# Autodesk Inventor assembly: Z Drive Assembly
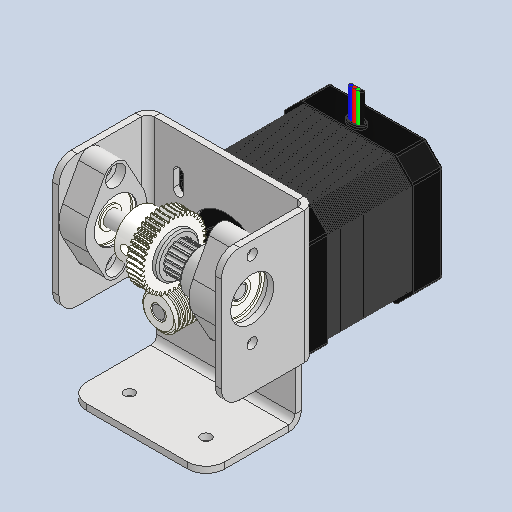
[picture p0: Inventor's stored thumbnail of the model, 512x512]
Saved by Autodesk Inventor 2022 (Build 260153000, 153)
## iProperties
Created: 2022-02-13
Part Number: Z Drive Assembly
Document SubType Name: Assembly
Designer: nicol
Author: nicol
## Documents named in this file (9)
- Z:\Projects\Bibble0\Z Drive Assembly.iam
- Z:\Projects\Bibble0\Sheet Metal\Z Drive Mount.ipt
- Z:\Projects\Bibble0\3D printed\Z Drive Bearing Holder.ipt
- Z:\Projects\Bibble0\Bearings\625 Bearing.ipt
- Z:\Projects\Bibble0\Hardware\5 x 50mm Shaft.ipt
- Z:\Projects\Bibble0\Hardware\GT2 Pulley 16T.ipt
- Z:\Projects\Bibble0\Hardware\METAL WORM GEAR_57545K624 v5.ipt
- Z:\Projects\Bibble0\Hardware\PLASTIC WORM GEAR_4037N115 v3.ipt
- Z:\Projects\Bibble0\Electronics\NEMA 17.ipt
## Components (10 placed, 8 different names)
1. Z Drive Mount:1 — Insert:4, Insert:5, Insert:6, Mate:5, Insert:8, Insert:9
2. Z Drive Bearing Holder:1 — Insert:4, Insert:5
3. Z Drive Bearing Holder:2 — Insert:6
4. 625 Bearing:1 — Mate:4
5. 625 Bearing:2
6. 5 x 50mm Shaft:1 — Mate:4
7. GT2 Pulley 16T:1
8. METAL WORM GEAR_57545K624 v5:1 — Insert:7
9. PLASTIC WORM GEAR_4037N115 v3:1
10. NEMA 17:1 — Mate:5, Insert:7, Insert:8, Insert:9
## Relationships (15: Insert 9, Mate 5, Flush 1)
- [Insert]: Z Drive Bearing Holder:2 ↔ 625 Bearing:1
- [Insert]: Z Drive Bearing Holder:1 ↔ 625 Bearing:2
- [Mate]: 625 Bearing:2 ↔ 5 x 50mm Shaft:1
- [Flush]: 625 Bearing:2 ↔ 5 x 50mm Shaft:1
- [Insert]: GT2 Pulley 16T:1 ↔ PLASTIC WORM GEAR_4037N115 v3:1
- [Mate] (15 mm): Z Drive Bearing Holder:1 ↔ PLASTIC WORM GEAR_4037N115 v3:1
- [Mate]: 5 x 50mm Shaft:1 ↔ PLASTIC WORM GEAR_4037N115 v3:1
- Mate:4: 625 Bearing:1 ↔ 5 x 50mm Shaft:1
- Insert:4: Z Drive Mount:1 ↔ Z Drive Bearing Holder:1
- Insert:5: Z Drive Mount:1 ↔ Z Drive Bearing Holder:1
- Insert:6: Z Drive Mount:1 ↔ Z Drive Bearing Holder:2
- Mate:5: Z Drive Mount:1 ↔ NEMA 17:1
- Insert:7: METAL WORM GEAR_57545K624 v5:1 ↔ NEMA 17:1
- Insert:8: Z Drive Mount:1 ↔ NEMA 17:1
- Insert:9: Z Drive Mount:1 ↔ NEMA 17:1
